# Autodesk Inventor assembly: VP STANDARD RAM ASSY
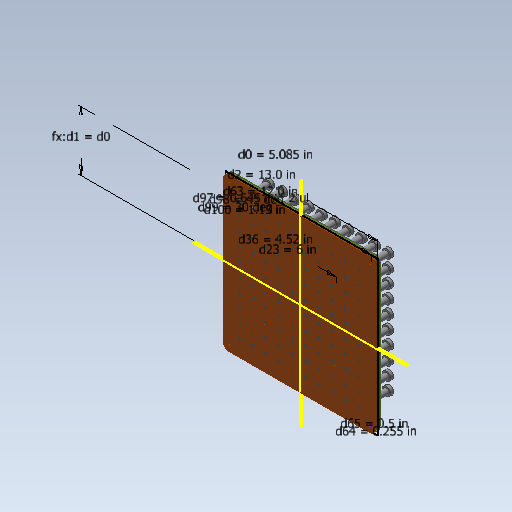
[picture p0: Inventor's stored thumbnail of the model, 512x512]
Saved by Autodesk Inventor 2020.3 (Build 243373000, 373)
## iProperties
RuleStatus: InUse
AfterDocSave0: file://Part Number Cleaner
Created: 2018-10-09
Vendor: HHMI: JRC - ID&F
Document SubType Name: Assembly
Designer: arnoldj
DESIGN DEPARTMENT: HHMI: JRC - ID&F
ALTERED ITEM PART NUMBER: N/A
ALTERED ITEM VENDOR: N/A
ALTERED ITEM DESCRIPTION: N/A
Author: arnoldj
Revision Number: 0
## Documents named in this file (8)
- C:\_WORKSPACE\DATA\PROJECTS\_PROJECTS BY LAB\FLY FACILITY\FLY MEDIA VIAL PLUGGING\VP STANDARD RAM ASSY.iam
- C:\_WORKSPACE\DATA\PROJECTS\_PROJECTS BY LAB\FLY FACILITY\FLY MEDIA VIAL PLUGGING\VP RAM NUT CAPTURE PLATE.ipt
- C:\_WORKSPACE\DATA\PROJECTS\_PROJECTS BY LAB\FLY FACILITY\FLY MEDIA VIAL PLUGGING\VP RAM PLATE.ipt
- C:\_WORKSPACE\DATA\COMMON\McMaster\MCMASTER 90633A009 8-32 LOCKNUT .ipt
- C:\_WORKSPACE\DATA\COMMON\McMaster\MCMASTER 94639A536_0_5D x 1L NYLON SPACER.ipt
- C:\_WORKSPACE\DATA\COMMON\McMaster\MCMASTER 94638A257_0_5D x 0_9375L NYLON SPACER.ipt
- C:\_WORKSPACE\DATA\COMMON\McMaster\MCMASTER 91771A207_8-32 x 2_5L FHMS SS.ipt
- C:\_WORKSPACE\DATA\PROJECTS\_PROJECTS BY LAB\FLY FACILITY\FLY MEDIA VIAL PLUGGING\VP RAM TIP.ipt
## Components (502 placed, 7 different names)
1. VP RAM PLATE:1 — Mate:1, Mate:2, Mate:3, Mate:4, Mate:5, Mate:6, Mate:7
2. VP RAM NUT CAPTURE PLATE:1 — Mate:1, Mate:2, Mate:3
3. VP RAM TIP:1 — Mate:13, Mate:14
4. MCMASTER 91771A207_8-32 x 2_5L FHMS SS:1
5. MCMASTER 94639A536_0_5D x 1L NYLON SPACER:1 — Mate:6, Mate:7
6. MCMASTER 94638A257_0_5D x 0_9375L NYLON SPACER:1 — Mate:13, Mate:14
7. MCMASTER 90633A009 8-32 LOCKNUT :1 — Mate:4, Mate:5
8. VP RAM TIP:2
9. MCMASTER 91771A207_8-32 x 2_5L FHMS SS:2
10. MCMASTER 94639A536_0_5D x 1L NYLON SPACER:2
11. MCMASTER 94638A257_0_5D x 0_9375L NYLON SPACER:2
12. MCMASTER 90633A009 8-32 LOCKNUT :2
13. VP RAM TIP:3
14. MCMASTER 91771A207_8-32 x 2_5L FHMS SS:3
15. MCMASTER 94639A536_0_5D x 1L NYLON SPACER:3
16. MCMASTER 94638A257_0_5D x 0_9375L NYLON SPACER:3
17. MCMASTER 90633A009 8-32 LOCKNUT :3
18. VP RAM TIP:4
19. MCMASTER 91771A207_8-32 x 2_5L FHMS SS:4
20. MCMASTER 94639A536_0_5D x 1L NYLON SPACER:4
21. MCMASTER 94638A257_0_5D x 0_9375L NYLON SPACER:4
22. MCMASTER 90633A009 8-32 LOCKNUT :4
23. VP RAM TIP:5
24. MCMASTER 91771A207_8-32 x 2_5L FHMS SS:5
25. MCMASTER 94639A536_0_5D x 1L NYLON SPACER:5
26. MCMASTER 94638A257_0_5D x 0_9375L NYLON SPACER:5
27. MCMASTER 90633A009 8-32 LOCKNUT :5
28. VP RAM TIP:6
29. MCMASTER 91771A207_8-32 x 2_5L FHMS SS:6
30. MCMASTER 94639A536_0_5D x 1L NYLON SPACER:6
31. MCMASTER 94638A257_0_5D x 0_9375L NYLON SPACER:6
32. MCMASTER 90633A009 8-32 LOCKNUT :6
33. VP RAM TIP:7
34. MCMASTER 91771A207_8-32 x 2_5L FHMS SS:7
35. MCMASTER 94639A536_0_5D x 1L NYLON SPACER:7
36. MCMASTER 94638A257_0_5D x 0_9375L NYLON SPACER:7
37. MCMASTER 90633A009 8-32 LOCKNUT :7
38. VP RAM TIP:8
39. MCMASTER 91771A207_8-32 x 2_5L FHMS SS:8
40. MCMASTER 94639A536_0_5D x 1L NYLON SPACER:8
41. MCMASTER 94638A257_0_5D x 0_9375L NYLON SPACER:8
42. MCMASTER 90633A009 8-32 LOCKNUT :8
43. VP RAM TIP:9
44. MCMASTER 91771A207_8-32 x 2_5L FHMS SS:9
45. MCMASTER 94639A536_0_5D x 1L NYLON SPACER:9
46. MCMASTER 94638A257_0_5D x 0_9375L NYLON SPACER:9
47. MCMASTER 90633A009 8-32 LOCKNUT :9
48. VP RAM TIP:10
49. MCMASTER 91771A207_8-32 x 2_5L FHMS SS:10
50. MCMASTER 94639A536_0_5D x 1L NYLON SPACER:10
51. MCMASTER 94638A257_0_5D x 0_9375L NYLON SPACER:10
52. MCMASTER 90633A009 8-32 LOCKNUT :10
53. VP RAM TIP:11
54. MCMASTER 91771A207_8-32 x 2_5L FHMS SS:11
55. MCMASTER 94639A536_0_5D x 1L NYLON SPACER:11
56. MCMASTER 94638A257_0_5D x 0_9375L NYLON SPACER:11
57. MCMASTER 90633A009 8-32 LOCKNUT :11
58. VP RAM TIP:12
59. MCMASTER 91771A207_8-32 x 2_5L FHMS SS:12
60. MCMASTER 94639A536_0_5D x 1L NYLON SPACER:12
61. MCMASTER 94638A257_0_5D x 0_9375L NYLON SPACER:12
62. MCMASTER 90633A009 8-32 LOCKNUT :12
63. VP RAM TIP:13
64. MCMASTER 91771A207_8-32 x 2_5L FHMS SS:13
65. MCMASTER 94639A536_0_5D x 1L NYLON SPACER:13
66. MCMASTER 94638A257_0_5D x 0_9375L NYLON SPACER:13
67. MCMASTER 90633A009 8-32 LOCKNUT :13
68. VP RAM TIP:14
69. MCMASTER 91771A207_8-32 x 2_5L FHMS SS:14
70. MCMASTER 94639A536_0_5D x 1L NYLON SPACER:14
71. MCMASTER 94638A257_0_5D x 0_9375L NYLON SPACER:14
72. MCMASTER 90633A009 8-32 LOCKNUT :14
73. VP RAM TIP:15
74. MCMASTER 91771A207_8-32 x 2_5L FHMS SS:15
75. MCMASTER 94639A536_0_5D x 1L NYLON SPACER:15
76. MCMASTER 94638A257_0_5D x 0_9375L NYLON SPACER:15
77. MCMASTER 90633A009 8-32 LOCKNUT :15
78. VP RAM TIP:16
79. MCMASTER 91771A207_8-32 x 2_5L FHMS SS:16
80. MCMASTER 94639A536_0_5D x 1L NYLON SPACER:16
81. MCMASTER 94638A257_0_5D x 0_9375L NYLON SPACER:16
82. MCMASTER 90633A009 8-32 LOCKNUT :16
83. VP RAM TIP:17
84. MCMASTER 91771A207_8-32 x 2_5L FHMS SS:17
85. MCMASTER 94639A536_0_5D x 1L NYLON SPACER:17
86. MCMASTER 94638A257_0_5D x 0_9375L NYLON SPACER:17
87. MCMASTER 90633A009 8-32 LOCKNUT :17
88. VP RAM TIP:18
89. MCMASTER 91771A207_8-32 x 2_5L FHMS SS:18
90. MCMASTER 94639A536_0_5D x 1L NYLON SPACER:18
91. MCMASTER 94638A257_0_5D x 0_9375L NYLON SPACER:18
92. MCMASTER 90633A009 8-32 LOCKNUT :18
93. VP RAM TIP:19
94. MCMASTER 91771A207_8-32 x 2_5L FHMS SS:19
95. MCMASTER 94639A536_0_5D x 1L NYLON SPACER:19
96. MCMASTER 94638A257_0_5D x 0_9375L NYLON SPACER:19
97. MCMASTER 90633A009 8-32 LOCKNUT :19
98. VP RAM TIP:20
99. MCMASTER 91771A207_8-32 x 2_5L FHMS SS:20
100. MCMASTER 94639A536_0_5D x 1L NYLON SPACER:20
101. MCMASTER 94638A257_0_5D x 0_9375L NYLON SPACER:20
102. MCMASTER 90633A009 8-32 LOCKNUT :20
103. VP RAM TIP:21
104. MCMASTER 91771A207_8-32 x 2_5L FHMS SS:21
105. MCMASTER 94639A536_0_5D x 1L NYLON SPACER:21
106. MCMASTER 94638A257_0_5D x 0_9375L NYLON SPACER:21
107. MCMASTER 90633A009 8-32 LOCKNUT :21
108. VP RAM TIP:22
109. MCMASTER 91771A207_8-32 x 2_5L FHMS SS:22
110. MCMASTER 94639A536_0_5D x 1L NYLON SPACER:22
111. MCMASTER 94638A257_0_5D x 0_9375L NYLON SPACER:22
112. MCMASTER 90633A009 8-32 LOCKNUT :22
113. VP RAM TIP:23
114. MCMASTER 91771A207_8-32 x 2_5L FHMS SS:23
115. MCMASTER 94639A536_0_5D x 1L NYLON SPACER:23
116. MCMASTER 94638A257_0_5D x 0_9375L NYLON SPACER:23
117. MCMASTER 90633A009 8-32 LOCKNUT :23
118. VP RAM TIP:24
119. MCMASTER 91771A207_8-32 x 2_5L FHMS SS:24
120. MCMASTER 94639A536_0_5D x 1L NYLON SPACER:24
121. MCMASTER 94638A257_0_5D x 0_9375L NYLON SPACER:24
122. MCMASTER 90633A009 8-32 LOCKNUT :24
123. VP RAM TIP:25
124. MCMASTER 91771A207_8-32 x 2_5L FHMS SS:25
125. MCMASTER 94639A536_0_5D x 1L NYLON SPACER:25
126. MCMASTER 94638A257_0_5D x 0_9375L NYLON SPACER:25
127. MCMASTER 90633A009 8-32 LOCKNUT :25
128. VP RAM TIP:26
129. MCMASTER 91771A207_8-32 x 2_5L FHMS SS:26
130. MCMASTER 94639A536_0_5D x 1L NYLON SPACER:26
131. MCMASTER 94638A257_0_5D x 0_9375L NYLON SPACER:26
132. MCMASTER 90633A009 8-32 LOCKNUT :26
133. VP RAM TIP:27
134. MCMASTER 91771A207_8-32 x 2_5L FHMS SS:27
135. MCMASTER 94639A536_0_5D x 1L NYLON SPACER:27
136. MCMASTER 94638A257_0_5D x 0_9375L NYLON SPACER:27
137. MCMASTER 90633A009 8-32 LOCKNUT :27
138. VP RAM TIP:28
139. MCMASTER 91771A207_8-32 x 2_5L FHMS SS:28
140. MCMASTER 94639A536_0_5D x 1L NYLON SPACER:28
141. MCMASTER 94638A257_0_5D x 0_9375L NYLON SPACER:28
142. MCMASTER 90633A009 8-32 LOCKNUT :28
143. VP RAM TIP:29
144. MCMASTER 91771A207_8-32 x 2_5L FHMS SS:29
145. MCMASTER 94639A536_0_5D x 1L NYLON SPACER:29
146. MCMASTER 94638A257_0_5D x 0_9375L NYLON SPACER:29
147. MCMASTER 90633A009 8-32 LOCKNUT :29
148. VP RAM TIP:30
149. MCMASTER 91771A207_8-32 x 2_5L FHMS SS:30
150. MCMASTER 94639A536_0_5D x 1L NYLON SPACER:30
151. MCMASTER 94638A257_0_5D x 0_9375L NYLON SPACER:30
152. MCMASTER 90633A009 8-32 LOCKNUT :30
153. VP RAM TIP:31
154. MCMASTER 91771A207_8-32 x 2_5L FHMS SS:31
155. MCMASTER 94639A536_0_5D x 1L NYLON SPACER:31
156. MCMASTER 94638A257_0_5D x 0_9375L NYLON SPACER:31
157. MCMASTER 90633A009 8-32 LOCKNUT :31
158. VP RAM TIP:32
159. MCMASTER 91771A207_8-32 x 2_5L FHMS SS:32
160. MCMASTER 94639A536_0_5D x 1L NYLON SPACER:32
161. MCMASTER 94638A257_0_5D x 0_9375L NYLON SPACER:32
162. MCMASTER 90633A009 8-32 LOCKNUT :32
163. VP RAM TIP:33
164. MCMASTER 91771A207_8-32 x 2_5L FHMS SS:33
165. MCMASTER 94639A536_0_5D x 1L NYLON SPACER:33
166. MCMASTER 94638A257_0_5D x 0_9375L NYLON SPACER:33
167. MCMASTER 90633A009 8-32 LOCKNUT :33
168. VP RAM TIP:34
169. MCMASTER 91771A207_8-32 x 2_5L FHMS SS:34
170. MCMASTER 94639A536_0_5D x 1L NYLON SPACER:34
171. MCMASTER 94638A257_0_5D x 0_9375L NYLON SPACER:34
172. MCMASTER 90633A009 8-32 LOCKNUT :34
173. VP RAM TIP:35
174. MCMASTER 91771A207_8-32 x 2_5L FHMS SS:35
175. MCMASTER 94639A536_0_5D x 1L NYLON SPACER:35
176. MCMASTER 94638A257_0_5D x 0_9375L NYLON SPACER:35
177. MCMASTER 90633A009 8-32 LOCKNUT :35
178. VP RAM TIP:36
179. MCMASTER 91771A207_8-32 x 2_5L FHMS SS:36
180. MCMASTER 94639A536_0_5D x 1L NYLON SPACER:36
181. MCMASTER 94638A257_0_5D x 0_9375L NYLON SPACER:36
182. MCMASTER 90633A009 8-32 LOCKNUT :36
183. VP RAM TIP:37
184. MCMASTER 91771A207_8-32 x 2_5L FHMS SS:37
185. MCMASTER 94639A536_0_5D x 1L NYLON SPACER:37
186. MCMASTER 94638A257_0_5D x 0_9375L NYLON SPACER:37
187. MCMASTER 90633A009 8-32 LOCKNUT :37
188. VP RAM TIP:38
189. MCMASTER 91771A207_8-32 x 2_5L FHMS SS:38
190. MCMASTER 94639A536_0_5D x 1L NYLON SPACER:38
191. MCMASTER 94638A257_0_5D x 0_9375L NYLON SPACER:38
192. MCMASTER 90633A009 8-32 LOCKNUT :38
193. VP RAM TIP:39
194. MCMASTER 91771A207_8-32 x 2_5L FHMS SS:39
195. MCMASTER 94639A536_0_5D x 1L NYLON SPACER:39
196. MCMASTER 94638A257_0_5D x 0_9375L NYLON SPACER:39
197. MCMASTER 90633A009 8-32 LOCKNUT :39
198. VP RAM TIP:40
199. MCMASTER 91771A207_8-32 x 2_5L FHMS SS:40
200. MCMASTER 94639A536_0_5D x 1L NYLON SPACER:40
201. MCMASTER 94638A257_0_5D x 0_9375L NYLON SPACER:40
202. MCMASTER 90633A009 8-32 LOCKNUT :40
203. VP RAM TIP:41
204. MCMASTER 91771A207_8-32 x 2_5L FHMS SS:41
205. MCMASTER 94639A536_0_5D x 1L NYLON SPACER:41
206. MCMASTER 94638A257_0_5D x 0_9375L NYLON SPACER:41
207. MCMASTER 90633A009 8-32 LOCKNUT :41
208. VP RAM TIP:42
209. MCMASTER 91771A207_8-32 x 2_5L FHMS SS:42
210. MCMASTER 94639A536_0_5D x 1L NYLON SPACER:42
211. MCMASTER 94638A257_0_5D x 0_9375L NYLON SPACER:42
212. MCMASTER 90633A009 8-32 LOCKNUT :42
213. VP RAM TIP:43
214. MCMASTER 91771A207_8-32 x 2_5L FHMS SS:43
215. MCMASTER 94639A536_0_5D x 1L NYLON SPACER:43
216. MCMASTER 94638A257_0_5D x 0_9375L NYLON SPACER:43
217. MCMASTER 90633A009 8-32 LOCKNUT :43
218. VP RAM TIP:44
219. MCMASTER 91771A207_8-32 x 2_5L FHMS SS:44
220. MCMASTER 94639A536_0_5D x 1L NYLON SPACER:44
221. MCMASTER 94638A257_0_5D x 0_9375L NYLON SPACER:44
222. MCMASTER 90633A009 8-32 LOCKNUT :44
223. VP RAM TIP:45
224. MCMASTER 91771A207_8-32 x 2_5L FHMS SS:45
225. MCMASTER 94639A536_0_5D x 1L NYLON SPACER:45
226. MCMASTER 94638A257_0_5D x 0_9375L NYLON SPACER:45
227. MCMASTER 90633A009 8-32 LOCKNUT :45
228. VP RAM TIP:46
229. MCMASTER 91771A207_8-32 x 2_5L FHMS SS:46
230. MCMASTER 94639A536_0_5D x 1L NYLON SPACER:46
231. MCMASTER 94638A257_0_5D x 0_9375L NYLON SPACER:46
232. MCMASTER 90633A009 8-32 LOCKNUT :46
233. VP RAM TIP:47
234. MCMASTER 91771A207_8-32 x 2_5L FHMS SS:47
235. MCMASTER 94639A536_0_5D x 1L NYLON SPACER:47
236. MCMASTER 94638A257_0_5D x 0_9375L NYLON SPACER:47
237. MCMASTER 90633A009 8-32 LOCKNUT :47
238. VP RAM TIP:48
239. MCMASTER 91771A207_8-32 x 2_5L FHMS SS:48
240. MCMASTER 94639A536_0_5D x 1L NYLON SPACER:48
241. MCMASTER 94638A257_0_5D x 0_9375L NYLON SPACER:48
242. MCMASTER 90633A009 8-32 LOCKNUT :48
243. VP RAM TIP:49
244. MCMASTER 91771A207_8-32 x 2_5L FHMS SS:49
245. MCMASTER 94639A536_0_5D x 1L NYLON SPACER:49
246. MCMASTER 94638A257_0_5D x 0_9375L NYLON SPACER:49
247. MCMASTER 90633A009 8-32 LOCKNUT :49
248. VP RAM TIP:50
249. MCMASTER 91771A207_8-32 x 2_5L FHMS SS:50
250. MCMASTER 94639A536_0_5D x 1L NYLON SPACER:50
251. MCMASTER 94638A257_0_5D x 0_9375L NYLON SPACER:50
252. MCMASTER 90633A009 8-32 LOCKNUT :50
253. VP RAM TIP:51
254. MCMASTER 91771A207_8-32 x 2_5L FHMS SS:51
255. MCMASTER 94639A536_0_5D x 1L NYLON SPACER:51
256. MCMASTER 94638A257_0_5D x 0_9375L NYLON SPACER:51
257. MCMASTER 90633A009 8-32 LOCKNUT :51
258. VP RAM TIP:52
259. MCMASTER 91771A207_8-32 x 2_5L FHMS SS:52
260. MCMASTER 94639A536_0_5D x 1L NYLON SPACER:52
261. MCMASTER 94638A257_0_5D x 0_9375L NYLON SPACER:52
262. MCMASTER 90633A009 8-32 LOCKNUT :52
263. VP RAM TIP:53
264. MCMASTER 91771A207_8-32 x 2_5L FHMS SS:53
265. MCMASTER 94639A536_0_5D x 1L NYLON SPACER:53
266. MCMASTER 94638A257_0_5D x 0_9375L NYLON SPACER:53
267. MCMASTER 90633A009 8-32 LOCKNUT :53
268. VP RAM TIP:54
269. MCMASTER 91771A207_8-32 x 2_5L FHMS SS:54
270. MCMASTER 94639A536_0_5D x 1L NYLON SPACER:54
271. MCMASTER 94638A257_0_5D x 0_9375L NYLON SPACER:54
272. MCMASTER 90633A009 8-32 LOCKNUT :54
273. VP RAM TIP:55
274. MCMASTER 91771A207_8-32 x 2_5L FHMS SS:55
275. MCMASTER 94639A536_0_5D x 1L NYLON SPACER:55
276. MCMASTER 94638A257_0_5D x 0_9375L NYLON SPACER:55
277. MCMASTER 90633A009 8-32 LOCKNUT :55
278. VP RAM TIP:56
279. MCMASTER 91771A207_8-32 x 2_5L FHMS SS:56
280. MCMASTER 94639A536_0_5D x 1L NYLON SPACER:56
281. MCMASTER 94638A257_0_5D x 0_9375L NYLON SPACER:56
282. MCMASTER 90633A009 8-32 LOCKNUT :56
283. VP RAM TIP:57
284. MCMASTER 91771A207_8-32 x 2_5L FHMS SS:57
285. MCMASTER 94639A536_0_5D x 1L NYLON SPACER:57
286. MCMASTER 94638A257_0_5D x 0_9375L NYLON SPACER:57
287. MCMASTER 90633A009 8-32 LOCKNUT :57
288. VP RAM TIP:58
289. MCMASTER 91771A207_8-32 x 2_5L FHMS SS:58
290. MCMASTER 94639A536_0_5D x 1L NYLON SPACER:58
291. MCMASTER 94638A257_0_5D x 0_9375L NYLON SPACER:58
292. MCMASTER 90633A009 8-32 LOCKNUT :58
293. VP RAM TIP:59
294. MCMASTER 91771A207_8-32 x 2_5L FHMS SS:59
295. MCMASTER 94639A536_0_5D x 1L NYLON SPACER:59
296. MCMASTER 94638A257_0_5D x 0_9375L NYLON SPACER:59
297. MCMASTER 90633A009 8-32 LOCKNUT :59
298. VP RAM TIP:60
299. MCMASTER 91771A207_8-32 x 2_5L FHMS SS:60
300. MCMASTER 94639A536_0_5D x 1L NYLON SPACER:60
301. MCMASTER 94638A257_0_5D x 0_9375L NYLON SPACER:60
302. MCMASTER 90633A009 8-32 LOCKNUT :60
303. VP RAM TIP:61
304. MCMASTER 91771A207_8-32 x 2_5L FHMS SS:61
305. MCMASTER 94639A536_0_5D x 1L NYLON SPACER:61
306. MCMASTER 94638A257_0_5D x 0_9375L NYLON SPACER:61
307. MCMASTER 90633A009 8-32 LOCKNUT :61
308. VP RAM TIP:62
309. MCMASTER 91771A207_8-32 x 2_5L FHMS SS:62
310. MCMASTER 94639A536_0_5D x 1L NYLON SPACER:62
311. MCMASTER 94638A257_0_5D x 0_9375L NYLON SPACER:62
312. MCMASTER 90633A009 8-32 LOCKNUT :62
313. VP RAM TIP:63
314. MCMASTER 91771A207_8-32 x 2_5L FHMS SS:63
315. MCMASTER 94639A536_0_5D x 1L NYLON SPACER:63
316. MCMASTER 94638A257_0_5D x 0_9375L NYLON SPACER:63
317. MCMASTER 90633A009 8-32 LOCKNUT :63
318. VP RAM TIP:64
319. MCMASTER 91771A207_8-32 x 2_5L FHMS SS:64
320. MCMASTER 94639A536_0_5D x 1L NYLON SPACER:64
321. MCMASTER 94638A257_0_5D x 0_9375L NYLON SPACER:64
322. MCMASTER 90633A009 8-32 LOCKNUT :64
323. VP RAM TIP:65
324. MCMASTER 91771A207_8-32 x 2_5L FHMS SS:65
325. MCMASTER 94639A536_0_5D x 1L NYLON SPACER:65
326. MCMASTER 94638A257_0_5D x 0_9375L NYLON SPACER:65
327. MCMASTER 90633A009 8-32 LOCKNUT :65
328. VP RAM TIP:66
329. MCMASTER 91771A207_8-32 x 2_5L FHMS SS:66
330. MCMASTER 94639A536_0_5D x 1L NYLON SPACER:66
331. MCMASTER 94638A257_0_5D x 0_9375L NYLON SPACER:66
332. MCMASTER 90633A009 8-32 LOCKNUT :66
333. VP RAM TIP:67
334. MCMASTER 91771A207_8-32 x 2_5L FHMS SS:67
335. MCMASTER 94639A536_0_5D x 1L NYLON SPACER:67
336. MCMASTER 94638A257_0_5D x 0_9375L NYLON SPACER:67
337. MCMASTER 90633A009 8-32 LOCKNUT :67
338. VP RAM TIP:68
339. MCMASTER 91771A207_8-32 x 2_5L FHMS SS:68
340. MCMASTER 94639A536_0_5D x 1L NYLON SPACER:68
341. MCMASTER 94638A257_0_5D x 0_9375L NYLON SPACER:68
342. MCMASTER 90633A009 8-32 LOCKNUT :68
343. VP RAM TIP:69
344. MCMASTER 91771A207_8-32 x 2_5L FHMS SS:69
345. MCMASTER 94639A536_0_5D x 1L NYLON SPACER:69
346. MCMASTER 94638A257_0_5D x 0_9375L NYLON SPACER:69
347. MCMASTER 90633A009 8-32 LOCKNUT :69
348. VP RAM TIP:70
349. MCMASTER 91771A207_8-32 x 2_5L FHMS SS:70
350. MCMASTER 94639A536_0_5D x 1L NYLON SPACER:70
351. MCMASTER 94638A257_0_5D x 0_9375L NYLON SPACER:70
352. MCMASTER 90633A009 8-32 LOCKNUT :70
353. VP RAM TIP:71
354. MCMASTER 91771A207_8-32 x 2_5L FHMS SS:71
355. MCMASTER 94639A536_0_5D x 1L NYLON SPACER:71
356. MCMASTER 94638A257_0_5D x 0_9375L NYLON SPACER:71
357. MCMASTER 90633A009 8-32 LOCKNUT :71
358. VP RAM TIP:72
359. MCMASTER 91771A207_8-32 x 2_5L FHMS SS:72
360. MCMASTER 94639A536_0_5D x 1L NYLON SPACER:72
361. MCMASTER 94638A257_0_5D x 0_9375L NYLON SPACER:72
362. MCMASTER 90633A009 8-32 LOCKNUT :72
363. VP RAM TIP:73
364. MCMASTER 91771A207_8-32 x 2_5L FHMS SS:73
365. MCMASTER 94639A536_0_5D x 1L NYLON SPACER:73
366. MCMASTER 94638A257_0_5D x 0_9375L NYLON SPACER:73
367. MCMASTER 90633A009 8-32 LOCKNUT :73
368. VP RAM TIP:74
369. MCMASTER 91771A207_8-32 x 2_5L FHMS SS:74
370. MCMASTER 94639A536_0_5D x 1L NYLON SPACER:74
371. MCMASTER 94638A257_0_5D x 0_9375L NYLON SPACER:74
372. MCMASTER 90633A009 8-32 LOCKNUT :74
373. VP RAM TIP:75
374. MCMASTER 91771A207_8-32 x 2_5L FHMS SS:75
375. MCMASTER 94639A536_0_5D x 1L NYLON SPACER:75
376. MCMASTER 94638A257_0_5D x 0_9375L NYLON SPACER:75
377. MCMASTER 90633A009 8-32 LOCKNUT :75
378. VP RAM TIP:76
379. MCMASTER 91771A207_8-32 x 2_5L FHMS SS:76
380. MCMASTER 94639A536_0_5D x 1L NYLON SPACER:76
381. MCMASTER 94638A257_0_5D x 0_9375L NYLON SPACER:76
382. MCMASTER 90633A009 8-32 LOCKNUT :76
383. VP RAM TIP:77
384. MCMASTER 91771A207_8-32 x 2_5L FHMS SS:77
385. MCMASTER 94639A536_0_5D x 1L NYLON SPACER:77
386. MCMASTER 94638A257_0_5D x 0_9375L NYLON SPACER:77
387. MCMASTER 90633A009 8-32 LOCKNUT :77
388. VP RAM TIP:78
389. MCMASTER 91771A207_8-32 x 2_5L FHMS SS:78
390. MCMASTER 94639A536_0_5D x 1L NYLON SPACER:78
391. MCMASTER 94638A257_0_5D x 0_9375L NYLON SPACER:78
392. MCMASTER 90633A009 8-32 LOCKNUT :78
393. VP RAM TIP:79
394. MCMASTER 91771A207_8-32 x 2_5L FHMS SS:79
395. MCMASTER 94639A536_0_5D x 1L NYLON SPACER:79
396. MCMASTER 94638A257_0_5D x 0_9375L NYLON SPACER:79
397. MCMASTER 90633A009 8-32 LOCKNUT :79
398. VP RAM TIP:80
399. MCMASTER 91771A207_8-32 x 2_5L FHMS SS:80
400. MCMASTER 94639A536_0_5D x 1L NYLON SPACER:80
401. MCMASTER 94638A257_0_5D x 0_9375L NYLON SPACER:80
402. MCMASTER 90633A009 8-32 LOCKNUT :80
403. VP RAM TIP:81
404. MCMASTER 91771A207_8-32 x 2_5L FHMS SS:81
405. MCMASTER 94639A536_0_5D x 1L NYLON SPACER:81
406. MCMASTER 94638A257_0_5D x 0_9375L NYLON SPACER:81
407. MCMASTER 90633A009 8-32 LOCKNUT :81
408. VP RAM TIP:82
409. MCMASTER 91771A207_8-32 x 2_5L FHMS SS:82
410. MCMASTER 94639A536_0_5D x 1L NYLON SPACER:82
411. MCMASTER 94638A257_0_5D x 0_9375L NYLON SPACER:82
412. MCMASTER 90633A009 8-32 LOCKNUT :82
413. VP RAM TIP:83
414. MCMASTER 91771A207_8-32 x 2_5L FHMS SS:83
415. MCMASTER 94639A536_0_5D x 1L NYLON SPACER:83
416. MCMASTER 94638A257_0_5D x 0_9375L NYLON SPACER:83
417. MCMASTER 90633A009 8-32 LOCKNUT :83
418. VP RAM TIP:84
419. MCMASTER 91771A207_8-32 x 2_5L FHMS SS:84
420. MCMASTER 94639A536_0_5D x 1L NYLON SPACER:84
421. MCMASTER 94638A257_0_5D x 0_9375L NYLON SPACER:84
422. MCMASTER 90633A009 8-32 LOCKNUT :84
423. VP RAM TIP:85
424. MCMASTER 91771A207_8-32 x 2_5L FHMS SS:85
425. MCMASTER 94639A536_0_5D x 1L NYLON SPACER:85
426. MCMASTER 94638A257_0_5D x 0_9375L NYLON SPACER:85
427. MCMASTER 90633A009 8-32 LOCKNUT :85
428. VP RAM TIP:86
429. MCMASTER 91771A207_8-32 x 2_5L FHMS SS:86
430. MCMASTER 94639A536_0_5D x 1L NYLON SPACER:86
431. MCMASTER 94638A257_0_5D x 0_9375L NYLON SPACER:86
432. MCMASTER 90633A009 8-32 LOCKNUT :86
433. VP RAM TIP:87
434. MCMASTER 91771A207_8-32 x 2_5L FHMS SS:87
435. MCMASTER 94639A536_0_5D x 1L NYLON SPACER:87
436. MCMASTER 94638A257_0_5D x 0_9375L NYLON SPACER:87
437. MCMASTER 90633A009 8-32 LOCKNUT :87
438. VP RAM TIP:88
439. MCMASTER 91771A207_8-32 x 2_5L FHMS SS:88
440. MCMASTER 94639A536_0_5D x 1L NYLON SPACER:88
441. MCMASTER 94638A257_0_5D x 0_9375L NYLON SPACER:88
442. MCMASTER 90633A009 8-32 LOCKNUT :88
443. VP RAM TIP:89
444. MCMASTER 91771A207_8-32 x 2_5L FHMS SS:89
445. MCMASTER 94639A536_0_5D x 1L NYLON SPACER:89
446. MCMASTER 94638A257_0_5D x 0_9375L NYLON SPACER:89
447. MCMASTER 90633A009 8-32 LOCKNUT :89
448. VP RAM TIP:90
449. MCMASTER 91771A207_8-32 x 2_5L FHMS SS:90
450. MCMASTER 94639A536_0_5D x 1L NYLON SPACER:90
451. MCMASTER 94638A257_0_5D x 0_9375L NYLON SPACER:90
452. MCMASTER 90633A009 8-32 LOCKNUT :90
453. VP RAM TIP:91
454. MCMASTER 91771A207_8-32 x 2_5L FHMS SS:91
455. MCMASTER 94639A536_0_5D x 1L NYLON SPACER:91
456. MCMASTER 94638A257_0_5D x 0_9375L NYLON SPACER:91
457. MCMASTER 90633A009 8-32 LOCKNUT :91
458. VP RAM TIP:92
459. MCMASTER 91771A207_8-32 x 2_5L FHMS SS:92
460. MCMASTER 94639A536_0_5D x 1L NYLON SPACER:92
461. MCMASTER 94638A257_0_5D x 0_9375L NYLON SPACER:92
462. MCMASTER 90633A009 8-32 LOCKNUT :92
463. VP RAM TIP:93
464. MCMASTER 91771A207_8-32 x 2_5L FHMS SS:93
465. MCMASTER 94639A536_0_5D x 1L NYLON SPACER:93
466. MCMASTER 94638A257_0_5D x 0_9375L NYLON SPACER:93
467. MCMASTER 90633A009 8-32 LOCKNUT :93
468. VP RAM TIP:94
469. MCMASTER 91771A207_8-32 x 2_5L FHMS SS:94
470. MCMASTER 94639A536_0_5D x 1L NYLON SPACER:94
471. MCMASTER 94638A257_0_5D x 0_9375L NYLON SPACER:94
472. MCMASTER 90633A009 8-32 LOCKNUT :94
473. VP RAM TIP:95
474. MCMASTER 91771A207_8-32 x 2_5L FHMS SS:95
475. MCMASTER 94639A536_0_5D x 1L NYLON SPACER:95
476. MCMASTER 94638A257_0_5D x 0_9375L NYLON SPACER:95
477. MCMASTER 90633A009 8-32 LOCKNUT :95
478. VP RAM TIP:96
479. MCMASTER 91771A207_8-32 x 2_5L FHMS SS:96
480. MCMASTER 94639A536_0_5D x 1L NYLON SPACER:96
481. MCMASTER 94638A257_0_5D x 0_9375L NYLON SPACER:96
482. MCMASTER 90633A009 8-32 LOCKNUT :96
483. VP RAM TIP:97
484. MCMASTER 91771A207_8-32 x 2_5L FHMS SS:97
485. MCMASTER 94639A536_0_5D x 1L NYLON SPACER:97
486. MCMASTER 94638A257_0_5D x 0_9375L NYLON SPACER:97
487. MCMASTER 90633A009 8-32 LOCKNUT :97
488. VP RAM TIP:98
489. MCMASTER 91771A207_8-32 x 2_5L FHMS SS:98
490. MCMASTER 94639A536_0_5D x 1L NYLON SPACER:98
491. MCMASTER 94638A257_0_5D x 0_9375L NYLON SPACER:98
492. MCMASTER 90633A009 8-32 LOCKNUT :98
493. VP RAM TIP:99
494. MCMASTER 91771A207_8-32 x 2_5L FHMS SS:99
495. MCMASTER 94639A536_0_5D x 1L NYLON SPACER:99
496. MCMASTER 94638A257_0_5D x 0_9375L NYLON SPACER:99
497. MCMASTER 90633A009 8-32 LOCKNUT :99
498. VP RAM TIP:100
499. MCMASTER 91771A207_8-32 x 2_5L FHMS SS:100
500. MCMASTER 94639A536_0_5D x 1L NYLON SPACER:100
501. MCMASTER 94638A257_0_5D x 0_9375L NYLON SPACER:100
502. MCMASTER 90633A009 8-32 LOCKNUT :100
## Component patterns: (100 elements, first: VP RAM TIP:1 + MCMASTER 91771A207_8-32 x 2_5L FHMS SS:1 + MCMASTER 94639A536_0_5D x 1L NYLON SPACER:1 + MCMASTER 94638A257_0_5D x 0_9375L NYLON SPACER:1 + MCMASTER 90633A009 8-32 LOCKNUT :1)
## Relationships (13: Mate 12, Flush 1)
- Mate:1: VP RAM PLATE:1 ↔ VP RAM NUT CAPTURE PLATE:1
- Mate:2: VP RAM PLATE:1 ↔ VP RAM NUT CAPTURE PLATE:1
- Mate:3: VP RAM PLATE:1 ↔ VP RAM NUT CAPTURE PLATE:1
- Mate:4: VP RAM PLATE:1 ↔ MCMASTER 90633A009 8-32 LOCKNUT :1
- Mate:5: VP RAM PLATE:1 ↔ MCMASTER 90633A009 8-32 LOCKNUT :1
- Mate:6: VP RAM PLATE:1 ↔ MCMASTER 94639A536_0_5D x 1L NYLON SPACER:1
- Mate:7: VP RAM PLATE:1 ↔ MCMASTER 94639A536_0_5D x 1L NYLON SPACER:1
- [Mate]: MCMASTER 94639A536_0_5D x 1L NYLON SPACER:1 ↔ MCMASTER 94638A257_0_5D x 0_9375L NYLON SPACER:1
- [Mate]: MCMASTER 94639A536_0_5D x 1L NYLON SPACER:1 ↔ MCMASTER 94638A257_0_5D x 0_9375L NYLON SPACER:1
- [Flush] (-3.81 mm): MCMASTER 91771A207_8-32 x 2_5L FHMS SS:1 ↔ MCMASTER 94638A257_0_5D x 0_9375L NYLON SPACER:1
- [Mate]: MCMASTER 91771A207_8-32 x 2_5L FHMS SS:1 ↔ MCMASTER 94638A257_0_5D x 0_9375L NYLON SPACER:1
- Mate:13: VP RAM TIP:1 ↔ MCMASTER 94638A257_0_5D x 0_9375L NYLON SPACER:1
- Mate:14: VP RAM TIP:1 ↔ MCMASTER 94638A257_0_5D x 0_9375L NYLON SPACER:1
